# Autodesk Inventor assembly: deskAssembly
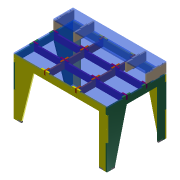
[picture p0: Inventor's stored thumbnail of the model, 180x180]
Saved by Autodesk Inventor 2015 SP1 (Build 190203100, 203)
## iProperties
Created: 2015-04-09
Part Number: deskAssembly
Document SubType Name: Assembly
Designer: Iain
Author: Iain
## Documents named in this file (9)
- D:\Users\Iain\Dropbox\FabAcademy\wk8_MakeSomethingBig\deskAssembly.iam
- D:\Users\Iain\Dropbox\FabAcademy\wk8_MakeSomethingBig\FrontLeg.ipt
- D:\Users\Iain\Dropbox\FabAcademy\wk8_MakeSomethingBig\SideLeg.ipt
- D:\Users\Iain\Dropbox\FabAcademy\wk8_MakeSomethingBig\longSlat.ipt
- D:\Users\Iain\Dropbox\FabAcademy\wk8_MakeSomethingBig\shortSlat.ipt
- D:\Users\Iain\Dropbox\FabAcademy\wk8_MakeSomethingBig\tableTop.ipt
- D:\Users\Iain\Dropbox\FabAcademy\wk8_MakeSomethingBig\shelfSide.ipt
- D:\Users\Iain\Dropbox\FabAcademy\wk8_MakeSomethingBig\shelfTop.ipt
- D:\Users\Iain\Dropbox\FabAcademy\wk8_MakeSomethingBig\foot.ipt
## Components (18 placed, 8 different names)
1. FrontLeg:1 — Flush:1, Flush:2, Flush:3, Flush:4, Flush:5, Flush:6, Flush:7, Flush:8, Flush:11, Flush:12, Flush:15, Flush:16, Flush:17, Flush:18, Mate:3, Mate:4, Flush:19, Flush:21, Flush:29, Flush:34, Flush:38
2. FrontLeg:2 — Flush:1, Flush:9, Flush:10, Flush:30, Flush:35, Flush:39
3. SideLeg:1 — Flush:3, Flush:4, Flush:7, Flush:8, Flush:9, Flush:10, Flush:20, Flush:31, Flush:32, Flush:37, Flush:40
4. SideLeg:2 — Flush:2, Flush:5, Flush:6, Flush:13, Flush:14, Mate:1, Mate:2, Flush:33, Flush:36
5. longSlat:1 — Flush:12, Flush:14, Mate:1
6. longSlat:2 — Flush:11, Flush:13, Mate:2
7. shortSlat:1 — Flush:16, Flush:18, Mate:3
8. shortSlat:2 — Flush:15, Flush:17, Mate:4
9. tableTop:1 — Flush:19, Flush:20, Flush:21, Mate:5, Mate:6, Mate:7, Mate:8, Flush:22, Flush:23, Flush:24, Flush:25, Mate:9, Mate:10, Mate:11, Mate:12, Flush:28
10. shelfSide:1 — Mate:7, Flush:25, Mate:12, Flush:26, Flush:27, Flush:28
11. shelfSide:2 — Mate:8, Flush:24, Mate:9, Mate:13
12. shelfSide:3 — Mate:5, Flush:22, Mate:10
13. shelfSide:4 — Mate:6, Flush:23, Mate:11
14. shelfTop:1 — Mate:13, Flush:26, Flush:27
15. foot:1 — Flush:29, Flush:33, Flush:34
16. foot:2 — Flush:31, Flush:35, Flush:36
17. foot:3 — Flush:30, Flush:37, Flush:38
18. foot:4 — Flush:32, Flush:39, Flush:40
## Relationships (53: Flush 40, Mate 13)
- Flush:1: FrontLeg:1 ↔ FrontLeg:2
- Flush:2: FrontLeg:1 ↔ SideLeg:2
- Flush:3: FrontLeg:1 ↔ SideLeg:1
- Flush:4: FrontLeg:1 ↔ SideLeg:1
- Flush:5: FrontLeg:1 ↔ SideLeg:2
- Flush:6: FrontLeg:1 ↔ SideLeg:2
- Flush:7: FrontLeg:1 ↔ SideLeg:1
- Flush:8: FrontLeg:1 ↔ SideLeg:1
- Flush:9: FrontLeg:2 ↔ SideLeg:1
- Flush:10: FrontLeg:2 ↔ SideLeg:1
- Flush:11: FrontLeg:1 ↔ longSlat:2
- Flush:12: FrontLeg:1 ↔ longSlat:1
- Flush:13: SideLeg:2 ↔ longSlat:2
- Flush:14: SideLeg:2 ↔ longSlat:1
- Mate:1: SideLeg:2 ↔ longSlat:1
- Mate:2: SideLeg:2 ↔ longSlat:2
- Flush:15: FrontLeg:1 ↔ shortSlat:2
- Flush:16: FrontLeg:1 ↔ shortSlat:1
- Flush:17: FrontLeg:1 ↔ shortSlat:2
- Flush:18: FrontLeg:1 ↔ shortSlat:1
- Mate:3: FrontLeg:1 ↔ shortSlat:1
- Mate:4: FrontLeg:1 ↔ shortSlat:2
- Flush:19: FrontLeg:1 ↔ tableTop:1
- Flush:20: SideLeg:1 ↔ tableTop:1
- Flush:21: FrontLeg:1 ↔ tableTop:1
- Mate:5: tableTop:1 ↔ shelfSide:3
- Mate:6: tableTop:1 ↔ shelfSide:4
- Mate:7: tableTop:1 ↔ shelfSide:1
- Mate:8: tableTop:1 ↔ shelfSide:2
- Flush:22: tableTop:1 ↔ shelfSide:3
- Flush:23: tableTop:1 ↔ shelfSide:4
- Flush:24: tableTop:1 ↔ shelfSide:2
- Flush:25: tableTop:1 ↔ shelfSide:1
- Mate:9: tableTop:1 ↔ shelfSide:2
- Mate:10: tableTop:1 ↔ shelfSide:3
- Mate:11: tableTop:1 ↔ shelfSide:4
- Mate:12: tableTop:1 ↔ shelfSide:1
- Mate:13: shelfSide:2 ↔ shelfTop:1
- Flush:26: shelfSide:1 ↔ shelfTop:1
- Flush:27: shelfSide:1 ↔ shelfTop:1
- Flush:28: tableTop:1 ↔ shelfSide:1
- Flush:29: FrontLeg:1 ↔ foot:1
- Flush:30: FrontLeg:2 ↔ foot:3
- Flush:31: SideLeg:1 ↔ foot:2
- Flush:32: SideLeg:1 ↔ foot:4
- Flush:33: SideLeg:2 ↔ foot:1
- Flush:34: FrontLeg:1 ↔ foot:1
- Flush:35: FrontLeg:2 ↔ foot:2
- Flush:36: SideLeg:2 ↔ foot:2
- Flush:37: SideLeg:1 ↔ foot:3
- Flush:38: FrontLeg:1 ↔ foot:3
- Flush:39: FrontLeg:2 ↔ foot:4
- Flush:40: SideLeg:1 ↔ foot:4
